# Autodesk Inventor assembly: !odom_pod
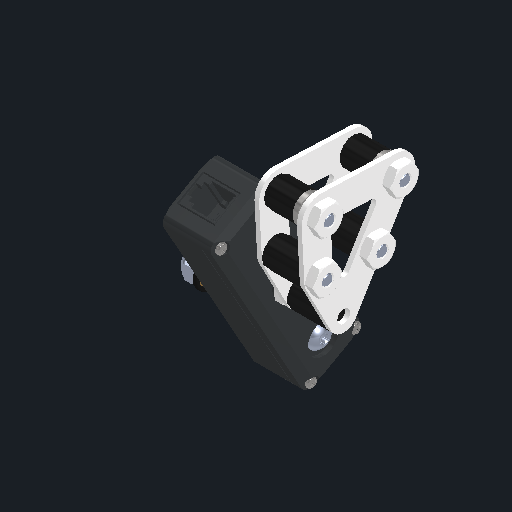
[picture p0: Inventor's stored thumbnail of the model, 512x512]
Saved by Autodesk Inventor 2025 (Build 290162000, 162)
## iProperties
Created: 2024-08-18
Part Number: !odom_pod
Document SubType Name: Assembly
Designer: averey
Author: averey
## Documents named in this file (18)
- D:\vex_robotics_high_stakes\hardware\cad\bots\ENIGMA\chassis\odom_pod\!odom_pod.iam
- C:\Users\avere\vex_robotics_high_stakes\hardware\cad\VEX-CAD-Inventor\Motion\Wheels\Omni Wheel\2.00 Omni AS, No Insert.ipt
- D:\vex_robotics_high_stakes\hardware\cad\VEX-CAD-Inventor\Electronics\Sensors\V5 Rotation Sensor.ipt
- C:\Users\avere\vex_robotics_high_stakes\hardware\cad\VEX-CAD-Inventor\Motion\Shaft HS\HS Spacer.ipt
- D:\vex_robotics_high_stakes\hardware\cad\VEX-CAD-Inventor\Motion\HS Shaft Adapter Circle.ipt
- D:\vex_robotics_high_stakes\hardware\cad\VEX-CAD-Inventor\Motion\Shaft HS\HS Spacer\HSpacer .0625.ipt
- D:\vex_robotics_high_stakes\hardware\cad\VEX-CAD-Inventor\Structure\Hardware\Screw Steel - Star\SScrew Star Smooth 1.750.ipt
- C:\Users\avere\vex_robotics_high_stakes\hardware\cad\VEX-CAD-Inventor\Structure\Hardware\Screw Steel - Star.ipt
- D:\vex_robotics_high_stakes\hardware\cad\VEX-CAD-Inventor\Structure\Hardware\Nut Thin Nylock.ipt
- D:\vex_robotics_high_stakes\hardware\cad\bots\ENIGMA\chassis\odom_pod\custom_parts\mount.ipt
- D:\vex_robotics_high_stakes\hardware\cad\VEX-CAD-Inventor\Motion\Spacers\Spacer Nylon .375 OD\NSpacer .375 OD x .375.ipt
- C:\Users\avere\vex_robotics_high_stakes\hardware\cad\VEX-CAD-Inventor\Motion\Spacers\Spacer Nylon .375 OD.ipt
- D:\vex_robotics_high_stakes\hardware\cad\VEX-CAD-Inventor\Motion\Spacers\Washer Steel\SWasher .375 OD x .062500.ipt
- C:\Users\avere\vex_robotics_high_stakes\hardware\cad\VEX-CAD-Inventor\Motion\Spacers\Washer Steel.ipt
- D:\vex_robotics_high_stakes\hardware\cad\VEX-CAD-Inventor\Motion\Spacers\Spacer Nylon .375 OD\NSpacer .375 OD x .500.ipt
- D:\vex_robotics_high_stakes\hardware\cad\VEX-CAD-Inventor\Structure\Hardware\Nut Nylon\Nut Nylon - White.ipt
- C:\Users\avere\vex_robotics_high_stakes\hardware\cad\VEX-CAD-Inventor\Structure\Hardware\Nut Nylon.ipt
- D:\vex_robotics_high_stakes\hardware\cad\VEX-CAD-Inventor\Structure\Hardware\Screw Steel - Star\SScrew Star Smooth .750.ipt
## Components (27 placed, 12 different names)
1. 2.00 Omni AS, No Insert:1 — Angle:1, Insert:12, Mate:2, Mate:3, Angle:2, Insert:32
2. V5 Rotation Sensor:1 — Angle:1, Insert:29, Mate:5, Mate:6, Mate:7, Flush:4, Insert:31
3. HSpacer .0625:1 — Insert:12, Mate:5, Mate:6, Mate:7
4. SScrew Star Smooth 1.750:1 — Insert:31
5. HS Shaft Adapter Circle:4 — Insert:13, Flush:3, Flush:4
6. HS Shaft Adapter Circle:5 — Insert:13, Flush:3, Mate:2, Mate:3, Insert:30
7. mount:1 — Insert:18, Mate:4, Insert:22, Insert:24, Insert:25, Insert:28, Insert:34, Insert:35, Insert:40, Insert:41
8. mount:2 — Insert:18, Mate:4, Insert:26, Insert:27, Insert:36, Insert:37, Insert:38, Insert:39
9. NSpacer .375 OD x .375:2 — Insert:22
10. SWasher .375 OD x .062500:2
11. NSpacer .375 OD x .375:3 — Insert:24
12. SWasher .375 OD x .062500:3
13. NSpacer .375 OD x .500:4 — Insert:26
14. NSpacer .375 OD x .500:5 — Insert:25
15. NSpacer .375 OD x .500:6 — Insert:27
16. Nut Nylon - White:1 — Insert:28, Insert:29
17. HS Shaft Adapter Circle:6 — Insert:30, Angle:2, Angle:3, Insert:33
18. HSpacer .0625:3 — Insert:32, Angle:3
19. Nut Thin Nylock:1 — Insert:33
20. SScrew Star Smooth .750:2 — Insert:34
21. SScrew Star Smooth .750:3 — Insert:35
22. Nut Nylon - White:2 — Insert:36
23. Nut Nylon - White:3 — Insert:37
24. Nut Nylon - White:4 — Insert:38
25. Nut Nylon - White:5 — Insert:39
26. SScrew Star Smooth .750:4 — Insert:41
27. SScrew Star Smooth .750:5 — Insert:40
## Relationships (35: Insert 24, Mate 6, Angle 3, Flush 2)
- Angle:1 (0 deg): 2.00 Omni AS, No Insert:1 ↔ V5 Rotation Sensor:1
- Insert:12: 2.00 Omni AS, No Insert:1 ↔ HSpacer .0625:1
- Insert:13: HS Shaft Adapter Circle:4 ↔ HS Shaft Adapter Circle:5
- Flush:3: HS Shaft Adapter Circle:4 ↔ HS Shaft Adapter Circle:5
- Mate:2: 2.00 Omni AS, No Insert:1 ↔ HS Shaft Adapter Circle:5
- Mate:3: 2.00 Omni AS, No Insert:1 ↔ HS Shaft Adapter Circle:5
- Insert:18 (12.7 mm): mount:1 ↔ mount:2
- Mate:4: mount:1 ↔ mount:2
- [Insert]: NSpacer .375 OD x .375:2 ↔ SWasher .375 OD x .062500:2
- Insert:22: mount:1 ↔ NSpacer .375 OD x .375:2
- [Insert]: NSpacer .375 OD x .375:3 ↔ SWasher .375 OD x .062500:3
- Insert:24: mount:1 ↔ NSpacer .375 OD x .375:3
- Insert:25: mount:1 ↔ NSpacer .375 OD x .500:5
- Insert:26: mount:2 ↔ NSpacer .375 OD x .500:4
- Insert:27: mount:2 ↔ NSpacer .375 OD x .500:6
- Insert:28: mount:1 ↔ Nut Nylon - White:1
- Insert:29: V5 Rotation Sensor:1 ↔ Nut Nylon - White:1
- Mate:5: V5 Rotation Sensor:1 ↔ HSpacer .0625:1
- Mate:6: V5 Rotation Sensor:1 ↔ HSpacer .0625:1
- Mate:7: V5 Rotation Sensor:1 ↔ HSpacer .0625:1
- Flush:4: V5 Rotation Sensor:1 ↔ HS Shaft Adapter Circle:4
- Insert:30: HS Shaft Adapter Circle:5 ↔ HS Shaft Adapter Circle:6
- Angle:2 (0 deg): 2.00 Omni AS, No Insert:1 ↔ HS Shaft Adapter Circle:6
- Insert:31: V5 Rotation Sensor:1 ↔ SScrew Star Smooth 1.750:1
- Insert:32: 2.00 Omni AS, No Insert:1 ↔ HSpacer .0625:3
- Angle:3 (0 deg): HS Shaft Adapter Circle:6 ↔ HSpacer .0625:3
- Insert:33: HS Shaft Adapter Circle:6 ↔ Nut Thin Nylock:1
- Insert:34: mount:1 ↔ SScrew Star Smooth .750:2
- Insert:35: mount:1 ↔ SScrew Star Smooth .750:3
- Insert:36: mount:2 ↔ Nut Nylon - White:2
- Insert:37: mount:2 ↔ Nut Nylon - White:3
- Insert:38: mount:2 ↔ Nut Nylon - White:4
- Insert:39: mount:2 ↔ Nut Nylon - White:5
- Insert:40: mount:1 ↔ SScrew Star Smooth .750:5
- Insert:41: mount:1 ↔ SScrew Star Smooth .750:4
## Named parameters: d40_d39 = 0 mm, d43_d39 = 0 mm
